# Autodesk Inventor assembly: AssemblyBase
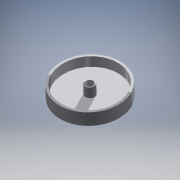
[picture p0: Inventor's stored thumbnail of the model, 180x180]
Saved by Autodesk Inventor 2017 (Build 210142000, 142)
## iProperties
Created: 2018-03-21
Part Number: AssemblyBase
Document SubType Name: Assembly
Designer: FablabGuest
Author: FablabGuest
## Documents named in this file (3)
- C:\Users\FablabGuest\Desktop\wheelhubcase\AssemblyBase.iam
- C:\Users\FablabGuest\Desktop\wheelhubcase\casept1.ipt
- C:\Users\FablabGuest\Desktop\wheelhubcase\casept2.ipt
## Components (2 placed, 2 different names)
1. casept1:1 — Rigid:1
2. casept2:1 — Rigid:1
## Relationships (1: WeldJoint 1)
- Rigid:1 [WeldJoint]: casept1:1 ↔ casept2:1
